# Autodesk Inventor assembly: XY Drive Subassy
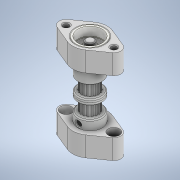
[picture p0: Inventor's stored thumbnail of the model, 180x180]
Saved by Autodesk Inventor 2022 (Build 260153000, 153)
## iProperties
Created: 2021-10-06
Part Number: XY Drive Subassy
Document SubType Name: Assembly
Designer: nicol
Author: nicol
## Documents named in this file (6)
- Z:\Projects\Bibble0\XY Drive Subassy.iam
- Z:\Projects\Bibble0\Bearings\625 Bearing.ipt
- Z:\Projects\Bibble0\3D printed\XY Drive Bearing Holder.ipt
- Z:\Projects\Bibble0\Hardware\GT2 Pulley 16T.ipt
- Z:\Projects\Bibble0\Hardware\5 x 50mm Shaft.ipt
- Z:\Projects\Bibble0\3D printed\Bearing Retaining Ring.ipt
## Components (9 placed, 5 different names)
1. 625 Bearing:1 — Insert:2, Insert:5, Insert:6, Insert:7
2. 625 Bearing:2 — Insert:1, Insert:3, Insert:8
3. XY Drive Bearing Holder:1 — Insert:1, Mate:1
4. XY Drive Bearing Holder:2 — Insert:2, Mate:1
5. GT2 Pulley 16T:1 — Insert:4, Insert:5
6. GT2 Pulley 16T:2 — Insert:3, Insert:4
7. 5 x 50mm Shaft:1 — Insert:6
8. Bearing Retaining Ring:1 — Insert:7
9. Bearing Retaining Ring:2 — Insert:8
## Relationships (9: Insert 8, Mate 1)
- Insert:1: 625 Bearing:2 ↔ XY Drive Bearing Holder:1
- Insert:2: 625 Bearing:1 ↔ XY Drive Bearing Holder:2
- Insert:3 (3 mm): 625 Bearing:2 ↔ GT2 Pulley 16T:2
- Insert:4: GT2 Pulley 16T:1 ↔ GT2 Pulley 16T:2
- Insert:5: 625 Bearing:1 ↔ GT2 Pulley 16T:1
- Insert:6 (-3 mm): 625 Bearing:1 ↔ 5 x 50mm Shaft:1
- Insert:7: 625 Bearing:1 ↔ Bearing Retaining Ring:1
- Insert:8: 625 Bearing:2 ↔ Bearing Retaining Ring:2
- Mate:1: XY Drive Bearing Holder:1 ↔ XY Drive Bearing Holder:2
